# Autodesk Inventor assembly: PLA_SetColor_d10_穴付き2
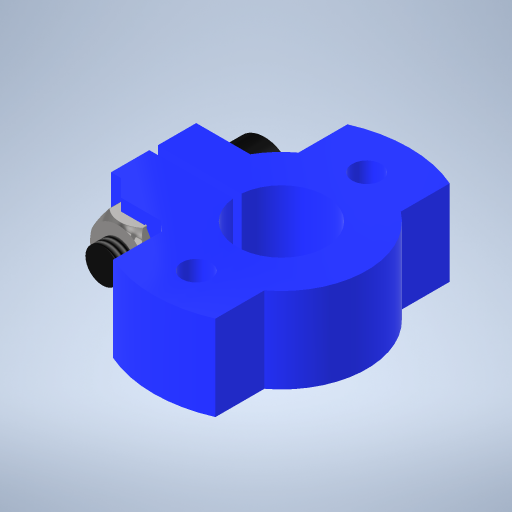
[picture p0: Inventor's stored thumbnail of the model, 512x512]
Saved by Autodesk Inventor 2023 (Build 270158000, 158)
## iProperties
Created: 2022-02-04
Part Number: PLA_SetColor_d10_穴付き2
Document SubType Name: Assembly
Designer: satot
Author: satot
## Documents named in this file (4)
- C:\Users\田之上巧太\Desktop\Basic_Parts\BasicParts\SetCollar\PLA_SetCollar_d10\PLA_SetColor_d10_穴付き.iam
- C:\Users\田之上巧太\Desktop\Basic_Parts\BasicParts\SetCollar\PLA_SetCollar_d10\PLA_SetColor_d10_穴付き.ipt
- C:\Users\田之上巧太\Desktop\Basic_Parts\BasicParts\SetCollar\PLA_SetCollar_d10\Bolt_M4_15_for_SetCollar_d10.ipt
- C:\Users\田之上巧太\Desktop\Basic_Parts\BasicParts\SetCollar\PLA_SetCollar_d10\Nut_M4_for_SetCollar.ipt
## Components (3 placed, 3 different names)
1. PLA_SetColor_d10_穴付き:1 — 回転:1, 回転:2
2. Bolt_M4_15_for_SetCollar_d10:1 — 回転:1
3. Nut_M4_for_SetCollar:1 — 回転:2
## Relationships (2: RevoluteJoint 2)
- 回転:1 [RevoluteJoint]: PLA_SetColor_d10_穴付き:1 ↔ Bolt_M4_15_for_SetCollar_d10:1
- 回転:2 [RevoluteJoint]: PLA_SetColor_d10_穴付き:1 ↔ Nut_M4_for_SetCollar:1
